# Autodesk Inventor assembly: legAssemblyV1
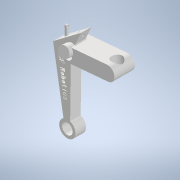
[picture p0: Inventor's stored thumbnail of the model, 180x180]
Saved by Autodesk Inventor 2022 (Build 260153000, 153)
## iProperties
Created: 2022-01-23
Part Number: legAssemblyV1
Document SubType Name: Assembly
Designer: money
Author: money
## Documents named in this file (4)
- C:\Users\money\Documents\Inventor\A2-Alternate-Mobility-Hand\legAssemblyV1.iam
- C:\Users\money\Documents\Inventor\A2-Alternate-Mobility-Hand\legV.1.ipt
- C:\Users\money\Documents\Inventor\A2-Alternate-Mobility-Hand\uperlegV1.ipt
- C:\Users\money\Documents\Inventor\A2-Alternate-Mobility-Hand\jointV0.ipt
## Components (3 placed, 3 different names)
1. legV.1:1 — Tangent:1
2. uperlegV1:1 — Tangent:2
3. jointV0:1 — Tangent:1, Tangent:2
## Relationships (2: Tangent 2)
- Tangent:1: legV.1:1 ↔ jointV0:1
- Tangent:2: uperlegV1:1 ↔ jointV0:1
